# Autodesk Inventor assembly: WR
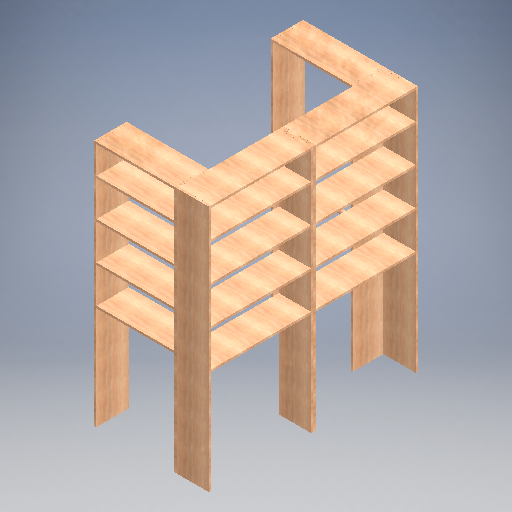
[picture p0: Inventor's stored thumbnail of the model, 512x512]
Saved by Autodesk Inventor 2025.2 (Build 292293000, 293)
## iProperties
Created: 2025-01-28
Part Number: WR
Document SubType Name: Assembly
Designer: Anna
Author: Anna
## Documents named in this file (15)
- E:\inventor\WRDRB\WARDROBE\WR.iam
- E:\inventor\WRDRB\WARDROBE\FLOOR.ipt
- E:\inventor\WRDRB\WARDROBE\LEFT WALL.ipt
- E:\inventor\WRDRB\WARDROBE\RIGHT WALL.ipt
- E:\inventor\WRDRB\WARDROBE\SH.1.ipt
- E:\inventor\WRDRB\WARDROBE\SH2.1.ipt
- E:\inventor\WRDRB\WARDROBE\PIPE.ipt
- E:\inventor\WRDRB\WARDROBE\PIPE LONG.ipt
- E:\inventor\WRDRB\WARDROBE\BACK WALL.ipt
- E:\inventor\WRDRB\WARDROBE\SIDE SH2.ipt
- E:\inventor\WRDRB\WARDROBE\WR\AIP\FEA\ezq3m2xmo.fins
- E:\inventor\WRDRB\WARDROBE\WR\AIP\FEA\ezq3m2xmo.fsat
- E:\inventor\WRDRB\WARDROBE\WR\AIP\FEA\ezq3m2xmo.ftes
- E:\inventor\WRDRB\WARDROBE\WR\AIP\FEA\ezq3m2xmo.fwiz
- E:\inventor\WRDRB\WARDROBE\WR\AIP\FEA\ezq3m2xuo.fmsh
## Components (30 placed, 9 different names)
1. FLOOR:1 — Flush:1, Flush:2, Mate:1, Flush:3, Mate:2, Mate:3, Flush:5, Flush:6, Flush:7, Flush:8, Flush:9, Flush:10, Flush:11, Mate:6, Mate:13, Mate:19, Flush:24, Mate:21, Flush:29, Mate:36
2. LEFT WALL:1 — Flush:1, Flush:2, Mate:1
3. RIGHT WALL:1 — Flush:3, Mate:2, Mate:3, Mate:22
4. BACK WALL:1 — Flush:24, Mate:21, Mate:22, Mate:23, Mate:32, Mate:34, Mate:35
5. SH.1:2 — Flush:6, Flush:7, Mate:5, Flush:13, Mate:7, Flush:14, Flush:15, Flush:17
6. SH.1:3 — Flush:8, Flush:9, Flush:12, Mate:4
7. SH.1:4 — Flush:5, Mate:19, Flush:31
8. SH.1:5 — Flush:10, Flush:11, Mate:12, Flush:23, Flush:30
9. SH2.1:1 — Flush:12, Mate:4
10. SH2.1:2 — Mate:5, Flush:13
11. SH2.1:3 — Mate:6, Mate:7, Flush:14, Flush:16, Mate:8
12. SH2.1:4 — Flush:15, Flush:16, Mate:8, Mate:9, Flush:18
13. SH2.1:5 — Mate:9, Flush:17, Flush:18, Mate:10, Flush:19
14. SH2.1:6 — Mate:10, Flush:19
15. PIPE:1 — Mate:11, Mate:12, Mate:13, Mate:18
16. PIPE LONG:1 — Flush:23, Mate:18
17. SIDE SH2:1 — Mate:23, Mate:37, Mate:38, Flush:32, Flush:36, Flush:37
18. SIDE SH2:2 — Mate:28, Flush:32, Flush:33
19. SIDE SH2:3 — Mate:28, Mate:31, Flush:25, Flush:33
20. SIDE SH2:4 — Mate:31, Mate:32, Flush:25, Mate:33, Flush:26, Flush:27
21. SIDE SH2:5 — Mate:33, Flush:26, Flush:27, Flush:46
22. SH.1:6 — Mate:35, Mate:36, Flush:31, Mate:37, Mate:38, Flush:34
23. SH.1:7 — Mate:34, Flush:29, Flush:30, Mate:43, Flush:45, Flush:50
24. SH.1:8 — Flush:35, Flush:36, Flush:37, Mate:39, Flush:38, Flush:39
25. SH.1:9 — Mate:39, Flush:38, Flush:39
26. SIDE SH2:6 — Flush:49, Flush:50
27. SIDE SH2:7 — Flush:48, Flush:49
28. SIDE SH2:8 — Flush:47, Flush:48
29. SIDE SH2:9 — Flush:47
30. SIDE SH2:10 — Mate:43, Flush:45, Flush:46
## Relationships (77: Flush 45, Mate 32)
- Flush:1: FLOOR:1 ↔ LEFT WALL:1
- Flush:2: FLOOR:1 ↔ LEFT WALL:1
- Mate:1: FLOOR:1 ↔ LEFT WALL:1
- Flush:3: FLOOR:1 ↔ RIGHT WALL:1
- Mate:2: FLOOR:1 ↔ RIGHT WALL:1
- Mate:3: FLOOR:1 ↔ RIGHT WALL:1
- Flush:5: FLOOR:1 ↔ SH.1:4
- Flush:6 (12.7 mm): FLOOR:1 ↔ SH.1:2
- Flush:7: FLOOR:1 ↔ SH.1:2
- Flush:8 (12.7 mm): FLOOR:1 ↔ SH.1:3
- Flush:9: FLOOR:1 ↔ SH.1:3
- Flush:10: FLOOR:1 ↔ SH.1:5
- Flush:11 (279.4 mm): FLOOR:1 ↔ SH.1:5
- Flush:12: SH.1:3 ↔ SH2.1:1
- Mate:4: SH.1:3 ↔ SH2.1:1
- Mate:5: SH.1:2 ↔ SH2.1:2
- Flush:13: SH.1:2 ↔ SH2.1:2
- Mate:6 (889 mm): FLOOR:1 ↔ SH2.1:3
- Mate:7: SH.1:2 ↔ SH2.1:3
- Flush:14: SH.1:2 ↔ SH2.1:3
- Flush:15: SH.1:2 ↔ SH2.1:4
- Flush:16: SH2.1:3 ↔ SH2.1:4
- Mate:8 (304.8 mm): SH2.1:3 ↔ SH2.1:4
- Mate:9 (304.8 mm): SH2.1:4 ↔ SH2.1:5
- Flush:17: SH.1:2 ↔ SH2.1:5
- Flush:18: SH2.1:4 ↔ SH2.1:5
- Mate:10 (304.8 mm): SH2.1:5 ↔ SH2.1:6
- Flush:19: SH2.1:5 ↔ SH2.1:6
- Mate:11: PIPE:1
- Mate:12: SH.1:5 ↔ PIPE:1
- Mate:13 (1016 mm): FLOOR:1 ↔ PIPE:1
- Flush:23: SH.1:5 ↔ PIPE LONG:1
- Mate:18 (1016 mm): PIPE:1 ↔ PIPE LONG:1
- Mate:19 (279.4 mm): FLOOR:1 ↔ SH.1:4
- Flush:24: FLOOR:1 ↔ BACK WALL:1
- Mate:21: FLOOR:1 ↔ BACK WALL:1
- Mate:22: RIGHT WALL:1 ↔ BACK WALL:1
- Mate:23: BACK WALL:1 ↔ SIDE SH2:1
- Mate:28 (304.8 mm): SIDE SH2:2 ↔ SIDE SH2:3
- Mate:31 (304.8 mm): SIDE SH2:3 ↔ SIDE SH2:4
- Mate:32: BACK WALL:1 ↔ SIDE SH2:4
- Flush:25: SIDE SH2:3 ↔ SIDE SH2:4
- Mate:33 (304.8 mm): SIDE SH2:4 ↔ SIDE SH2:5
- Flush:26: SIDE SH2:4 ↔ SIDE SH2:5
- Flush:27: SIDE SH2:4 ↔ SIDE SH2:5
- Mate:34: BACK WALL:1 ↔ SH.1:7
- Flush:29: FLOOR:1 ↔ SH.1:7
- Flush:30: SH.1:5 ↔ SH.1:7
- Mate:35: BACK WALL:1 ↔ SH.1:6
- Mate:36: FLOOR:1 ↔ SH.1:6
- Flush:31: SH.1:4 ↔ SH.1:6
- Mate:37: SIDE SH2:1 ↔ SH.1:6
- Mate:38: SIDE SH2:1 ↔ SH.1:6
- Flush:32: SIDE SH2:1 ↔ SIDE SH2:2
- Flush:33: SIDE SH2:2 ↔ SIDE SH2:3
- Flush:34 (-901.7 mm): SH.1:6
- Flush:35: SH.1:8
- Flush:36: SIDE SH2:1 ↔ SH.1:8
- Flush:37: SIDE SH2:1 ↔ SH.1:8
- Mate:39: SH.1:8 ↔ SH.1:9
- Flush:38: SH.1:8 ↔ SH.1:9
- Flush:39: SH.1:8 ↔ SH.1:9
- [Mate] (304.8 mm): SIDE SH2:7 ↔ SIDE SH2:8
- [Mate] (304.8 mm): SIDE SH2:8 ↔ SIDE SH2:9
- [Flush]: SIDE SH2:8 ↔ SIDE SH2:9
- [Mate] (304.8 mm): SIDE SH2:9 ↔ SIDE SH2:10
- [Flush]: SIDE SH2:9 ↔ SIDE SH2:10
- [Flush]: SIDE SH2:9 ↔ SIDE SH2:10
- [Flush]: SIDE SH2:6 ↔ SIDE SH2:7
- [Flush]: SIDE SH2:7 ↔ SIDE SH2:8
- Mate:43: SH.1:7 ↔ SIDE SH2:10
- Flush:45: SH.1:7 ↔ SIDE SH2:10
- Flush:46: SIDE SH2:5 ↔ SIDE SH2:10
- Flush:47: SIDE SH2:8 ↔ SIDE SH2:9
- Flush:48: SIDE SH2:7 ↔ SIDE SH2:8
- Flush:49: SIDE SH2:6 ↔ SIDE SH2:7
- Flush:50: SH.1:7 ↔ SIDE SH2:6
## Named parameters: d111_d87 = 304.8 mm, d112_d88 = 0 mm, d113_d89 = 0 mm, d114_d81 = 304.8 mm, d115_d84 = 304.8 mm, d116_d86 = 0 mm, d117_d102 = 0 mm, d118_d103 = 0 mm
